# Autodesk Inventor assembly: DoubleCross_SymWiden_testasm
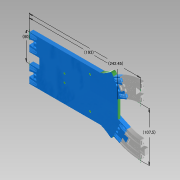
[picture p0: Inventor's stored thumbnail of the model, 180x180]
Saved by Autodesk Inventor 2021 (Build 250183000, 183)
## iProperties
Created: 2021-03-07
Part Number: DoubleCross_SymWiden_testasm
Document SubType Name: Assembly
Designer: kumagai
Author: kumagai
## Documents named in this file (4)
- X:\Develop\CAD\PlaRails\DoubleCross\DoubleCross_SymWiden_testasm.iam
- X:\Develop\CAD\PlaRails\DoubleCross\DoubleCross_SymWiden_C.ipt
- X:\Develop\CAD\PlaRails\CurveRail\CurveRail\CurveRail-89-25.ipt
- X:\Develop\CAD\PlaRails\CurveRail\CurveRail.ipt
## Components (3 placed, 2 different names)
1. DoubleCross_SymWiden_C:1 — フラッシュ:1, フラッシュ:2, メイト:1, メイト:2, メイト:3, メイト:4
2. CurveRail-89-25:1 — フラッシュ:1, メイト:1, メイト:2
3. CurveRail-89-25:2 — フラッシュ:2, メイト:3, メイト:4
## Relationships (6: Mate 4, Flush 2)
- フラッシュ:1 [Flush]: DoubleCross_SymWiden_C:1 ↔ CurveRail-89-25:1
- フラッシュ:2 [Flush]: DoubleCross_SymWiden_C:1 ↔ CurveRail-89-25:2
- メイト:1 [Mate]: DoubleCross_SymWiden_C:1 ↔ CurveRail-89-25:1
- メイト:2 [Mate]: DoubleCross_SymWiden_C:1 ↔ CurveRail-89-25:1
- メイト:3 [Mate]: DoubleCross_SymWiden_C:1 ↔ CurveRail-89-25:2
- メイト:4 [Mate]: DoubleCross_SymWiden_C:1 ↔ CurveRail-89-25:2
